# Autodesk Inventor assembly: CPS_002_Versa+775Motor
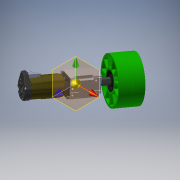
[picture p0: Inventor's stored thumbnail of the model, 180x180]
Saved by Autodesk Inventor 2018 (Build 220112000, 112)
## iProperties
Created: 2020-01-30
Part Number: CPS_002_Versa+775Motor
Document SubType Name: Assembly
Designer: 22turnmaxw
Author: 22turnmaxw
## Documents named in this file (4)
- C:\Users\jd2\Documents\GrabCAD\Infinite Recharge 2020\Build season\CPS_002_Versa+775Motor.iam
- C:\Users\jd2\Documents\GrabCAD\Infinite Recharge 2020\Brainstorming\Versaplanetary\775 Motor.ipt
- C:\Users\jd2\Documents\GrabCAD\Infinite Recharge 2020\Brainstorming\Versaplanetary\VersaPlanetary Gearbox.iam
- C:\Users\jd2\Documents\GrabCAD\Infinite Recharge 2020\Build season\CPS_005_GreenWheel.iam
## Components (4 placed, 3 different names)
1. 775 Motor:1 — Mate:1, Mate:2, Angle:1
2. VersaPlanetary Gearbox:1 [sub-assembly] — Mate:1, Mate:2, Angle:1, Flush:1, Mate:3, Mate:4, Mate:5, Mate:6, Flush:2
3. CPS_005_GreenWheel:1 [sub-assembly] — Flush:1, Mate:3, Mate:4
4. CPS_005_GreenWheel:2 [sub-assembly] — Mate:5, Mate:6, Flush:2
## Relationships (9: Mate 6, Flush 2, Angle 1)
- Mate:1: 775 Motor:1 ↔ VersaPlanetary Gearbox:1
- Mate:2: 775 Motor:1 ↔ VersaPlanetary Gearbox:1
- Angle:1 (0 deg): 775 Motor:1 ↔ VersaPlanetary Gearbox:1
- Flush:1 (-25.4 mm): VersaPlanetary Gearbox:1 ↔ CPS_005_GreenWheel:1
- Mate:3: VersaPlanetary Gearbox:1 ↔ CPS_005_GreenWheel:1
- Mate:4: VersaPlanetary Gearbox:1 ↔ CPS_005_GreenWheel:1
- Mate:5: VersaPlanetary Gearbox:1 ↔ CPS_005_GreenWheel:2
- Mate:6: VersaPlanetary Gearbox:1 ↔ CPS_005_GreenWheel:2
- Flush:2: VersaPlanetary Gearbox:1 ↔ CPS_005_GreenWheel:2
